# Autodesk Inventor assembly: Assembly2
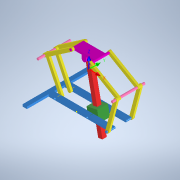
[picture p0: Inventor's stored thumbnail of the model, 180x180]
Saved by Autodesk Inventor 2022 (Build 260153000, 153)
## iProperties
Created: 2022-01-15
Part Number: Assembly2
Document SubType Name: Assembly
Designer: G S SHOURIE
Mass: 6843.83 g
Surface Area: 2470.18 cm^2
Volume: 855.478 cm^3
Density: 8 g/cm^3
Author: G S SHOURIE
## Documents named in this file (18)
- C:\Users\G S SHOURIE\Desktop\SHOURIE\IMPORTANT STUFF\Ecole Centrale de Nantes\Masters\Studies\Design of Robots\GRAMA SRINIVAS SHOURIE\Model for Inventor\constrainedAssembly.iam
- C:\Users\G S SHOURIE\Desktop\SHOURIE\IMPORTANT STUFF\Ecole Centrale de Nantes\Masters\Studies\Design of Robots\GRAMA SRINIVAS SHOURIE\Model for Inventor\base.ipt
- C:\Users\G S SHOURIE\Desktop\SHOURIE\IMPORTANT STUFF\Ecole Centrale de Nantes\Masters\Studies\Design of Robots\GRAMA SRINIVAS SHOURIE\Model for Inventor\innerLink.ipt
- C:\Users\G S SHOURIE\Desktop\SHOURIE\IMPORTANT STUFF\Ecole Centrale de Nantes\Masters\Studies\Design of Robots\GRAMA SRINIVAS SHOURIE\Model for Inventor\outerLink.ipt
- C:\Users\G S SHOURIE\Desktop\SHOURIE\IMPORTANT STUFF\Ecole Centrale de Nantes\Masters\Studies\Design of Robots\GRAMA SRINIVAS SHOURIE\Model for Inventor\prismaticFulcrum.ipt
- C:\Users\G S SHOURIE\Desktop\SHOURIE\IMPORTANT STUFF\Ecole Centrale de Nantes\Masters\Studies\Design of Robots\GRAMA SRINIVAS SHOURIE\Model for Inventor\prismaticLink.ipt
- C:\Users\G S SHOURIE\Desktop\SHOURIE\IMPORTANT STUFF\Ecole Centrale de Nantes\Masters\Studies\Design of Robots\GRAMA SRINIVAS SHOURIE\Model for Inventor\endEffector.ipt
- C:\Users\G S SHOURIE\Desktop\SHOURIE\IMPORTANT STUFF\Ecole Centrale de Nantes\Masters\Studies\Design of Robots\GRAMA SRINIVAS SHOURIE\Model for Inventor\pin.ipt
- C:\Users\G S SHOURIE\Desktop\SHOURIE\IMPORTANT STUFF\Ecole Centrale de Nantes\Masters\Studies\Design of Robots\GRAMA SRINIVAS SHOURIE\Model for Inventor\pathBase.ipt
- C:\Users\G S SHOURIE\Desktop\SHOURIE\IMPORTANT STUFF\Ecole Centrale de Nantes\Masters\Studies\Design of Robots\GRAMA SRINIVAS SHOURIE\Model for Inventor\pathFollower.ipt
- C:\Users\G S SHOURIE\Desktop\SHOURIE\IMPORTANT STUFF\Ecole Centrale de Nantes\Masters\Studies\Design of Robots\GRAMA SRINIVAS SHOURIE\Model for Inventor\constrainedAssembly\AIP\FEA\dusb5kdpc.fins
- C:\Users\G S SHOURIE\Desktop\SHOURIE\IMPORTANT STUFF\Ecole Centrale de Nantes\Masters\Studies\Design of Robots\GRAMA SRINIVAS SHOURIE\Model for Inventor\constrainedAssembly\AIP\FEA\dusb5kdq8.fsat
- C:\Users\G S SHOURIE\Desktop\SHOURIE\IMPORTANT STUFF\Ecole Centrale de Nantes\Masters\Studies\Design of Robots\GRAMA SRINIVAS SHOURIE\Model for Inventor\constrainedAssembly\AIP\FEA\dusb5kdq8.ftes
- C:\Users\G S SHOURIE\Desktop\SHOURIE\IMPORTANT STUFF\Ecole Centrale de Nantes\Masters\Studies\Design of Robots\GRAMA SRINIVAS SHOURIE\Model for Inventor\constrainedAssembly\AIP\FEA\dusb5kdq8.fwiz
- C:\Users\G S SHOURIE\Desktop\SHOURIE\IMPORTANT STUFF\Ecole Centrale de Nantes\Masters\Studies\Design of Robots\GRAMA SRINIVAS SHOURIE\Model for Inventor\constrainedAssembly\AIP\FEA\dusb5ke00.fmsh
- C:\Users\G S SHOURIE\Desktop\SHOURIE\IMPORTANT STUFF\Ecole Centrale de Nantes\Masters\Studies\Design of Robots\GRAMA SRINIVAS SHOURIE\Model for Inventor\constrainedAssembly\AIP\FEA\dusruz2e8.fres
- C:\Users\G S SHOURIE\Desktop\SHOURIE\IMPORTANT STUFF\Ecole Centrale de Nantes\Masters\Studies\Design of Robots\GRAMA SRINIVAS SHOURIE\Model for Inventor\constrainedAssembly\AIP\FEA\dusruz2xs.fmsh
- C:\Users\G S SHOURIE\Desktop\SHOURIE\IMPORTANT STUFF\Ecole Centrale de Nantes\Masters\Studies\Design of Robots\GRAMA SRINIVAS SHOURIE\Model for Inventor\constrainedAssembly\AIP\FEA\dusruz2xt.fres
## Components (16 placed, 9 different names)
1. base:1 — Mate:1, Mate:2, Mate:3, Mate:4, Mate:5, Mate:6, Mate:7, Mate:8, Mate:9, Mate:10
2. innerLink:1 — Mate:3, Mate:4, Mate:13, Mate:14
3. innerLink:2 — Mate:1, Mate:2, Mate:15, Mate:16, Mate:22
4. outerLink:1 — Mate:5, Mate:6, Mate:19, Mate:20
5. outerLink:2 — Mate:7, Mate:8, Mate:17, Mate:18, Mate:21, Mate:29, Flush:1
6. prismaticFulcrum:1 — Mate:9, Mate:10, Mate:11, Mate:12
7. prismaticLink:1 — Mate:11, Mate:12, Mate:27
8. outerLink:3 — Mate:19, Mate:20, Mate:21, Mate:26
9. outerLink:4 — Mate:17, Mate:18, Mate:25
10. outerLink:5 — Mate:13, Mate:14, Mate:22, Mate:24, Mate:30, Flush:2
11. outerLink:6 — Mate:15, Mate:16, Mate:23, Mate:28
12. endEffector:1 — Mate:23, Mate:24, Mate:25, Mate:26, Mate:27, Mate:28, Mate:36, Angle:2
13. pin:1 — Mate:29, Flush:1
14. pin:2 — Mate:30, Flush:2
15. pathBase:1 — Mate:31, Mate:34, Mate:35, Tangent:1, Tangent:2
16. pathFollower:1 — Mate:35, Tangent:1, Tangent:2, Angle:1, Mate:36
## Relationships (43: Mate 36, Flush 3, Tangent 2, Angle 2)
- Mate:1: base:1 ↔ innerLink:2
- Mate:2: base:1 ↔ innerLink:2
- Mate:3: base:1 ↔ innerLink:1
- Mate:4: base:1 ↔ innerLink:1
- Mate:5: base:1 ↔ outerLink:1
- Mate:6: base:1 ↔ outerLink:1
- Mate:7: base:1 ↔ outerLink:2
- Mate:8: base:1 ↔ outerLink:2
- Mate:9: base:1 ↔ prismaticFulcrum:1
- Mate:10: base:1 ↔ prismaticFulcrum:1
- Mate:11: prismaticFulcrum:1 ↔ prismaticLink:1
- Mate:12: prismaticFulcrum:1 ↔ prismaticLink:1
- Mate:13: innerLink:1 ↔ outerLink:5
- Mate:14: innerLink:1 ↔ outerLink:5
- Mate:15: innerLink:2 ↔ outerLink:6
- Mate:16: innerLink:2 ↔ outerLink:6
- Mate:17: outerLink:2 ↔ outerLink:4
- Mate:18: outerLink:2 ↔ outerLink:4
- Mate:19: outerLink:1 ↔ outerLink:3
- Mate:20: outerLink:1 ↔ outerLink:3
- Mate:21: outerLink:2 ↔ outerLink:3
- Mate:22: innerLink:2 ↔ outerLink:5
- Mate:23: outerLink:6 ↔ endEffector:1
- Mate:24: outerLink:5 ↔ endEffector:1
- Mate:25: outerLink:4 ↔ endEffector:1
- Mate:26: outerLink:3 ↔ endEffector:1
- Mate:27: prismaticLink:1 ↔ endEffector:1
- Mate:28: outerLink:6 ↔ endEffector:1
- Mate:29: outerLink:2 ↔ pin:1
- Flush:1 (-15 mm): outerLink:2 ↔ pin:1
- Mate:30: outerLink:5 ↔ pin:2
- Flush:2 (-50 mm): outerLink:5 ↔ pin:2
- Flush:3 (200 mm)
- Mate:31: pathBase:1
- Mate:32
- Mate:33
- Mate:34: pathBase:1
- Mate:35: pathBase:1 ↔ pathFollower:1
- Tangent:1: pathBase:1 ↔ pathFollower:1
- Tangent:2: pathBase:1 ↔ pathFollower:1
- Angle:1 (270 deg): pathFollower:1
- Mate:36: endEffector:1 ↔ pathFollower:1
- Angle:2 (180 deg): endEffector:1
